# Autodesk Inventor assembly: intake
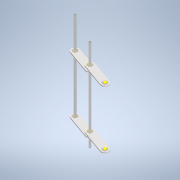
[picture p0: Inventor's stored thumbnail of the model, 180x180]
Saved by Autodesk Inventor 2022 (Build 260153000, 153)
## iProperties
Created: 2023-01-10
Part Number: intake
Document SubType Name: Assembly
Designer: s135320
Author: s135320
## Documents named in this file (4)
- D:\intake.iam
- D:\intake-2.ipt
- D:\intake-1.ipt
- D:\STEP Files\Bearings\1-2inch Hex Bering\217-3875-STEP-20140818.ipt
## Components (14 placed, 3 different names)
1. intake-2:1 — Mate:5, Mate:6, Mate:7, Mate:8
2. intake-2:2 — Mate:9, Mate:10, Mate:11, Mate:12, Mate:17, Mate:18, Mate:19, Mate:20
3. intake-1:1 — Mate:1, Flush:1, Mate:2, Flush:2
4. 217-3875-STEP-20140818:2 — Mate:2, Flush:2, Mate:10, Mate:11
5. 217-3875-STEP-20140818:3 — Mate:1, Flush:1, Mate:7, Mate:8
6. intake-1:3
7. 217-3875-STEP-20140818:5 — Mate:9, Mate:12
8. 217-3875-STEP-20140818:6 — Mate:5, Mate:6
9. intake-1:4
10. 217-3875-STEP-20140818:7
11. 217-3875-STEP-20140818:8 — Mate:17, Mate:18
12. intake-1:5
13. 217-3875-STEP-20140818:9
14. 217-3875-STEP-20140818:10 — Mate:19, Mate:20
## Relationships (28: Mate 20, Flush 8)
- Mate:1: intake-1:1 ↔ 217-3875-STEP-20140818:3
- Flush:1: intake-1:1 ↔ 217-3875-STEP-20140818:3
- Mate:2: intake-1:1 ↔ 217-3875-STEP-20140818:2
- Flush:2: intake-1:1 ↔ 217-3875-STEP-20140818:2
- [Mate]: intake-1:3 ↔ 217-3875-STEP-20140818:6
- [Flush]: intake-1:3 ↔ 217-3875-STEP-20140818:6
- [Mate]: intake-1:3 ↔ 217-3875-STEP-20140818:5
- [Flush]: intake-1:3 ↔ 217-3875-STEP-20140818:5
- Mate:5: intake-2:1 ↔ 217-3875-STEP-20140818:6
- Mate:6: intake-2:1 ↔ 217-3875-STEP-20140818:6
- Mate:7: intake-2:1 ↔ 217-3875-STEP-20140818:3
- Mate:8: intake-2:1 ↔ 217-3875-STEP-20140818:3
- Mate:9: intake-2:2 ↔ 217-3875-STEP-20140818:5
- Mate:10: intake-2:2 ↔ 217-3875-STEP-20140818:2
- Mate:11: intake-2:2 ↔ 217-3875-STEP-20140818:2
- Mate:12: intake-2:2 ↔ 217-3875-STEP-20140818:5
- [Mate]: intake-1:4 ↔ 217-3875-STEP-20140818:8
- [Flush]: intake-1:4 ↔ 217-3875-STEP-20140818:8
- [Mate]: intake-1:4 ↔ 217-3875-STEP-20140818:7
- [Flush]: intake-1:4 ↔ 217-3875-STEP-20140818:7
- [Mate]: intake-1:5 ↔ 217-3875-STEP-20140818:10
- [Flush]: intake-1:5 ↔ 217-3875-STEP-20140818:10
- [Mate]: intake-1:5 ↔ 217-3875-STEP-20140818:9
- [Flush]: intake-1:5 ↔ 217-3875-STEP-20140818:9
- Mate:17: intake-2:2 ↔ 217-3875-STEP-20140818:8
- Mate:18: intake-2:2 ↔ 217-3875-STEP-20140818:8
- Mate:19: intake-2:2 ↔ 217-3875-STEP-20140818:10
- Mate:20: intake-2:2 ↔ 217-3875-STEP-20140818:10
## Named parameters: d4_d0 = 0 mm, d5_d1 = 0 mm, d6_d2 = 0 mm, d7_d3 = 0 mm, d16_d4_d0 = 0 mm, d17_d5_d1 = 0 mm, d18_d6_d2 = 0 mm, d19_d7_d3 = 0 mm, d20_d4_d0 = 0 mm, d21_d5_d1 = 0 mm, d22_d6_d2 = 0 mm, d23_d7_d3 = 0 mm
